# Autodesk Inventor assembly: Loop Assembly
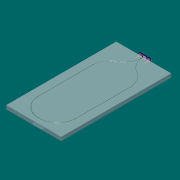
[picture p0: Inventor's stored thumbnail of the model, 180x180]
Saved by Autodesk Inventor 2016 (Build 200138000, 138)
## iProperties
Created: 2015-08-17
Part Number: Loop Assembly
Document SubType Name: Assembly
Designer: Cosmic
Author: Cosmic
## Documents named in this file (8)
- C:\Users\Sawaiz\OneDrive\projects\scintillatorPanel\loopLargePanel.iam
- C:\Users\Sawaiz\OneDrive\projects\scintillatorPanel\loopLargePanel.ipt
- C:\Users\Sawaiz\OneDrive\projects\scintillatorPanel\fiberLargeLoop.ipt
- C:\Users\Sawaiz\OneDrive\projects\scintillatorPanel\m3Washer.ipt
- C:\Users\Sawaiz\OneDrive\projects\scintillatorPanel\2mmSpacer.ipt
- C:\Users\Sawaiz\OneDrive\projects\scintillatorPanel\mppcSensorInterface\cad\sensor.iam
- C:\Users\Sawaiz\OneDrive\projects\scintillatorPanel\m3x8.ipt
- C:\Users\Sawaiz\OneDrive\projects\scintillatorPanel\Scintillator.xlsx
## Components (9 placed, 6 different names)
1. loopLargePanel:1 — Flush:1, Tangent:1, Tangent:2, Tangent:3, Flush:2, Mate:12, Mate:13, Mate:14, Flush:4, Mate:15, Mate:16, Mate:20, Mate:21
2. fiberLargeLoop:1 — Flush:1, Tangent:1, Tangent:2, Tangent:3, Flush:2, Flush:4, Mate:15, Mate:16
3. m3Washer:1 — Mate:1, Mate:2, Mate:25
4. m3Washer:2 — Mate:3, Mate:4
5. 2mmSpacer:1 — Mate:1, Mate:2, Mate:10, Mate:14, Mate:18
6. 2mmSpacer:2 — Mate:3, Mate:4, Mate:11, Mate:17
7. sensor:1 [sub-assembly] — Mate:22, Mate:23, Mate:24, Mate:25
8. m3x8:1 — Flush:3, Mate:10, Mate:12, Mate:17, Flush:5, Mate:21, Mate:24
9. m3x8:2 — Flush:3, Mate:11, Mate:13, Mate:18, Flush:5, Mate:20, Mate:22, Mate:23
## Relationships (27: Mate 19, Flush 5, Tangent 3)
- Flush:1: loopLargePanel:1 ↔ fiberLargeLoop:1
- Tangent:1 (0.15 mm): loopLargePanel:1 ↔ fiberLargeLoop:1
- Tangent:2 (0.15 mm): loopLargePanel:1 ↔ fiberLargeLoop:1
- Tangent:3 (0.15 mm): loopLargePanel:1 ↔ fiberLargeLoop:1
- Flush:2: loopLargePanel:1 ↔ fiberLargeLoop:1
- Mate:1: m3Washer:1 ↔ 2mmSpacer:1
- Mate:2: m3Washer:1 ↔ 2mmSpacer:1
- Mate:3: m3Washer:2 ↔ 2mmSpacer:2
- Mate:4: m3Washer:2 ↔ 2mmSpacer:2
- Flush:3: m3x8:1 ↔ m3x8:2
- Mate:10: 2mmSpacer:1 ↔ m3x8:1
- Mate:11: 2mmSpacer:2 ↔ m3x8:2
- Mate:12: loopLargePanel:1 ↔ m3x8:1
- Mate:13: loopLargePanel:1 ↔ m3x8:2
- Mate:14: loopLargePanel:1 ↔ 2mmSpacer:1
- Flush:4: loopLargePanel:1 ↔ fiberLargeLoop:1
- Mate:15 (0.15 mm): loopLargePanel:1 ↔ fiberLargeLoop:1
- Mate:16 (0.15 mm): loopLargePanel:1 ↔ fiberLargeLoop:1
- Mate:17: 2mmSpacer:2 ↔ m3x8:1
- Mate:18: 2mmSpacer:1 ↔ m3x8:2
- Flush:5: m3x8:1 ↔ m3x8:2
- Mate:20: loopLargePanel:1 ↔ m3x8:2
- Mate:21: loopLargePanel:1 ↔ m3x8:1
- Mate:22: sensor:1 ↔ m3x8:2
- Mate:23: sensor:1 ↔ m3x8:2
- Mate:24: sensor:1 ↔ m3x8:1
- Mate:25: m3Washer:1 ↔ sensor:1
## Named parameters: OpticalFiberClearence = 0.15 mm, MPPCClearence = 0.075 mm, FiberSensorClerence = 0.5 mm, OpticalFiberDiameter = 1 mm, ScintillatorThickness = 10 mm, SmallTrackDiameter = 175 mm, LargeTrackRatio = 3, ScintillatorEdgeClearence = 3 mm, ScintillatorWidth = 145 mm, ScintillatorHeight = 290 mm, ShallowTrackDepth = 1.3 mm, MPPCSensorClearence = 1.45 mm, MPPCSensorOffsett = 2.105 mm, MPPCWidth = 5.9 mm, MPPCHeight = 6.55 mm, FiberEdgeOffsett = 5 mm, MPPCDepth = 1 mm, LongFiberAngle = 30 deg, ShortFiberAngle = 78 deg, LoopLargeTrackRatio = 1.1, LoopSmallTrackDiameter = 90 mm, MountingScrewDepth = 2 mm, MountingScrewOffsett = 12 mm, LoopLength = 140 mm
